# Autodesk Inventor assembly: Model-2
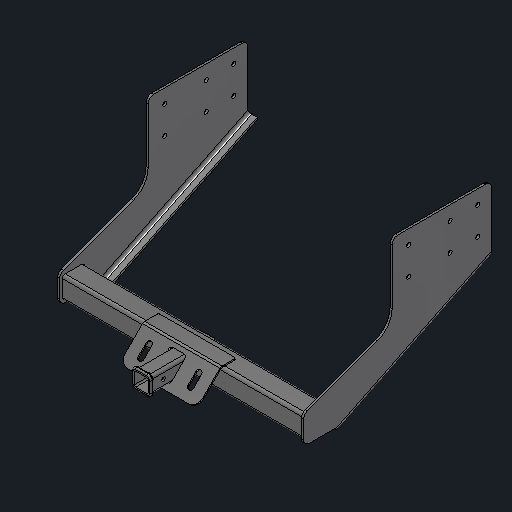
[picture p0: Inventor's stored thumbnail of the model, 512x512]
Saved by Autodesk Inventor 2025.1 (Build 291241000, 241)
## iProperties
Created: 2026-02-13
Part Number: Model-2
Document SubType Name: Assembly
Designer: Desktop -24
Mass: 20583.6 g
Surface Area: 8150.6 cm^2
Volume: 2573.11 cm^3
Density: 7.99949 g/cm^3
encoded128: ÌStandard (in)rÎ
Family: ASSEMBLY
Author: Desktop -24
## Documents named in this file (6)
- F:\OneDrive - nLeague Technologies Private Limited\Desktop\Sharath Chandra\Rear Hitch\Model-2\Model-2.iam
- F:\OneDrive - nLeague Technologies Private Limited\Desktop\Sharath Chandra\Rear Hitch\Model-2\Model-2_Base Tube-1.ipt
- F:\OneDrive - nLeague Technologies Private Limited\Desktop\Sharath Chandra\Rear Hitch\Model-2\Model-2_Sheet-LH.ipt
- F:\OneDrive - nLeague Technologies Private Limited\Desktop\Sharath Chandra\Rear Hitch\Model-2\Model-2_Sheet-RH.ipt
- F:\OneDrive - nLeague Technologies Private Limited\Desktop\Sharath Chandra\Rear Hitch\Model-2\Model-2_Base Tube-2.ipt
- F:\OneDrive - nLeague Technologies Private Limited\Desktop\Sharath Chandra\Rear Hitch\Model-2\Model-2_Sheet Stifferner.ipt
## Components (5 placed, 5 different names)
1. Model-2_Base Tube-1:1 — Mate:4, Mate:5, Flush:2, Mate:6, Flush:3, Flush:4, Mate:7, Flush:5, Mate:10, Flush:7, Mate:11
2. Model-2_Base Tube-2:1 — Mate:4, Mate:5, Flush:2
3. Model-2_Sheet-LH:1 — Mate:6, Flush:3, Flush:4, Flush:6
4. Model-2_Sheet-RH:1 — Mate:7, Flush:5, Flush:6
5. Model-2_Sheet Stifferner:1 — Mate:10, Flush:7, Mate:11
## Relationships (12: Mate 6, Flush 6)
- Mate:4: Model-2_Base Tube-1:1 ↔ Model-2_Base Tube-2:1
- Mate:5: Model-2_Base Tube-1:1 ↔ Model-2_Base Tube-2:1
- Flush:2 (9.525 mm): Model-2_Base Tube-1:1 ↔ Model-2_Base Tube-2:1
- Mate:6: Model-2_Base Tube-1:1 ↔ Model-2_Sheet-LH:1
- Flush:3 (12.7 mm): Model-2_Base Tube-1:1 ↔ Model-2_Sheet-LH:1
- Flush:4 (12.7 mm): Model-2_Base Tube-1:1 ↔ Model-2_Sheet-LH:1
- Mate:7: Model-2_Base Tube-1:1 ↔ Model-2_Sheet-RH:1
- Flush:5 (-12.7 mm): Model-2_Base Tube-1:1 ↔ Model-2_Sheet-RH:1
- Flush:6: Model-2_Sheet-LH:1 ↔ Model-2_Sheet-RH:1
- Mate:10: Model-2_Base Tube-1:1 ↔ Model-2_Sheet Stifferner:1
- Flush:7 (-38.1 mm): Model-2_Base Tube-1:1 ↔ Model-2_Sheet Stifferner:1
- Mate:11: Model-2_Base Tube-1:1 ↔ Model-2_Sheet Stifferner:1
